# Autodesk Inventor assembly: b4
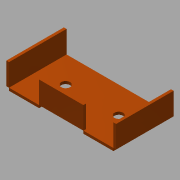
[picture p0: Inventor's stored thumbnail of the model, 180x180]
Saved by Autodesk Inventor 2016 (Build 200138000, 138)
## iProperties
Created: 2016-06-11
Part Number: b4
Document SubType Name: Assembly
Designer: daniel
Author: daniel
## Documents named in this file (4)
- C:\Users\daniel\Documents\GitHub\cardboard-stage-metric\stage\b4.iam
- C:\Users\daniel\Documents\GitHub\cardboard-stage-metric\stage\b3b.ipt
- C:\Users\daniel\Documents\GitHub\cardboard-stage-metric\stage\b3c.ipt
- C:\Users\daniel\Documents\GitHub\cardboard-stage-metric\stage\b4a.ipt
## Components (4 placed, 3 different names)
1. b4a:1 — Mate:1, Mate:2, Mate:3, Mate:4, Mate:5, Flush:1, Flush:2, Mate:6, Mate:7
2. b3b:1 — Mate:4, Mate:5, Flush:1
3. b3c:1 — Mate:1, Mate:2, Mate:3
4. b3b:2 — Flush:2, Mate:6, Mate:7
## Relationships (9: Mate 7, Flush 2)
- Mate:1: b4a:1 ↔ b3c:1
- Mate:2: b4a:1 ↔ b3c:1
- Mate:3: b4a:1 ↔ b3c:1
- Mate:4: b4a:1 ↔ b3b:1
- Mate:5: b4a:1 ↔ b3b:1
- Flush:1: b4a:1 ↔ b3b:1
- Flush:2: b4a:1 ↔ b3b:2
- Mate:6: b4a:1 ↔ b3b:2
- Mate:7: b4a:1 ↔ b3b:2
